# Autodesk Inventor assembly: Assembly1
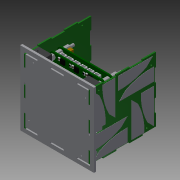
[picture p0: Inventor's stored thumbnail of the model, 180x180]
Saved by Autodesk Inventor 2015 SP1 (Build 190203100, 203)
## iProperties
Created: 2015-08-25
Part Number: Assembly1
Document SubType Name: Assembly
Designer: Kartikye
Author: Kartikye
## Documents named in this file (11)
- C:\Users\Kartikye\Documents\GitHub\SASSat\Structure\V5\Assembly1.iam
- C:\Users\Kartikye\Documents\GitHub\SASSat\Structure\V5\Bottom Panel.ipt
- C:\Users\Kartikye\Documents\GitHub\SASSat\Structure\V5\Corner2.ipt
- C:\Users\Kartikye\Documents\GitHub\SASSat\Structure\V5\Side Solar Panel.iam
- C:\Users\Kartikye\Documents\GitHub\SASSat\Structure\Imported Components\D2MQ_1\D2MQ_1.iam
- C:\Users\Kartikye\Documents\GitHub\SASSat\Structure\V5\Side Solar Panel with Switch.iam
- C:\Users\Kartikye\Documents\GitHub\SASSat\Structure\V5\Corner Switch Holder.ipt
- C:\Users\Kartikye\Documents\GitHub\SASSat\Structure\EPS\PQ60 EPS FV4.brd.iam
- C:\Users\Kartikye\Documents\GitHub\SASSat\Structure\Standoff.ipt
- C:\Users\Kartikye\Documents\GitHub\SASSat\Structure\Radio\PQ60 Radio FV1.brd.iam
- C:\Users\Kartikye\Documents\GitHub\SASSat\Structure\m1.6.ipt
## Components (31 placed, 10 different names)
1. Bottom Panel:1 — Mate:25, Mate:26, Mate:27, Mate:28, Mate:29, Mate:30, Mate:31, Mate:38, Mate:40
2. Corner Switch Holder:2 — Mate:26, Mate:36, Mate:37, Insert:1, Insert:16
3. Corner2:2 — Mate:28, Mate:34, Mate:35, Insert:2
4. Corner Switch Holder:1 — Mate:29, Mate:32, Mate:33, Mate:42, Insert:18, Insert:19
5. Corner2:4 — Mate:23, Mate:24, Mate:27, Insert:5
6. Side Solar Panel:1 [sub-assembly] — Mate:13, Mate:14, Flush:1, Mate:15, Mate:16, Flush:2, Mate:32, Mate:34
7. Side Solar Panel with Switch:2 [sub-assembly] — Mate:15, Mate:16, Flush:2, Mate:17, Mate:18, Mate:19, Flush:3, Mate:24, Mate:33, Flush:5, Mate:41, Insert:22
8. Side Solar Panel:3 [sub-assembly] — Mate:17, Mate:18, Mate:19, Flush:3, Mate:23, Mate:25, Mate:30, Mate:36
9. Side Solar Panel with Switch:1 [sub-assembly] — Mate:13, Mate:14, Flush:1, Mate:31, Mate:35, Mate:37, Mate:39, Flush:4, Insert:20
10. D2MQ_1:1 [sub-assembly] — Mate:38, Mate:39, Flush:4, Insert:21
11. D2MQ_1:2 [sub-assembly] — Mate:40, Flush:5, Mate:41
12. PQ60 EPS FV4.brd:1 [sub-assembly] — Insert:3, Insert:4, Insert:6, Insert:7, Insert:8, Insert:9
13. Standoff:1 — Insert:8
14. Standoff:2 — Insert:9, Insert:11
15. Standoff:3 — Insert:1
16. Standoff:4 — Insert:5
17. Standoff:5 — Mate:42, Insert:4
18. Standoff:6 — Insert:6
19. Standoff:7 — Insert:7, Insert:10
20. Standoff:8 — Insert:2, Insert:3
21. PQ60 Radio FV1.brd:1 [sub-assembly] — Insert:10, Insert:11, Insert:12, Insert:13, Insert:14, Insert:15
22. Standoff:9 — Insert:12
23. Standoff:10 — Insert:15
24. Standoff:11 — Insert:13
25. Standoff:12 — Insert:14
26. m1.6:1 — Insert:19
27. m1.6:2 — Insert:18
28. m1.6:3 — Insert:21
29. m1.6:4 — Insert:16
30. m1.6:5 — Insert:22
31. m1.6:6 — Insert:20
## Relationships (53: Mate 27, Insert 21, Flush 5)
- Mate:13: Side Solar Panel:1 ↔ Side Solar Panel with Switch:1
- Mate:14: Side Solar Panel:1 ↔ Side Solar Panel with Switch:1
- Flush:1: Side Solar Panel:1 ↔ Side Solar Panel with Switch:1
- Mate:15: Side Solar Panel:1 ↔ Side Solar Panel with Switch:2
- Mate:16: Side Solar Panel:1 ↔ Side Solar Panel with Switch:2
- Flush:2: Side Solar Panel:1 ↔ Side Solar Panel with Switch:2
- Mate:17: Side Solar Panel with Switch:2 ↔ Side Solar Panel:3
- Mate:18: Side Solar Panel with Switch:2 ↔ Side Solar Panel:3
- Mate:19: Side Solar Panel with Switch:2 ↔ Side Solar Panel:3
- Flush:3: Side Solar Panel with Switch:2 ↔ Side Solar Panel:3
- Mate:23: Corner2:4 ↔ Side Solar Panel:3
- Mate:24: Corner2:4 ↔ Side Solar Panel with Switch:2
- Mate:25: Bottom Panel:1 ↔ Side Solar Panel:3
- Mate:26: Bottom Panel:1 ↔ Corner Switch Holder:2
- Mate:27: Bottom Panel:1 ↔ Corner2:4
- Mate:28: Bottom Panel:1 ↔ Corner2:2
- Mate:29: Bottom Panel:1 ↔ Corner Switch Holder:1
- Mate:30: Bottom Panel:1 ↔ Side Solar Panel:3
- Mate:31: Bottom Panel:1 ↔ Side Solar Panel with Switch:1
- Mate:32: Corner Switch Holder:1 ↔ Side Solar Panel:1
- Mate:33: Corner Switch Holder:1 ↔ Side Solar Panel with Switch:2
- Mate:34: Corner2:2 ↔ Side Solar Panel:1
- Mate:35: Corner2:2 ↔ Side Solar Panel with Switch:1
- Mate:36: Corner Switch Holder:2 ↔ Side Solar Panel:3
- Mate:37: Corner Switch Holder:2 ↔ Side Solar Panel with Switch:1
- Mate:38: Bottom Panel:1 ↔ D2MQ_1:1
- Mate:39: Side Solar Panel with Switch:1 ↔ D2MQ_1:1
- Flush:4: Side Solar Panel with Switch:1 ↔ D2MQ_1:1
- Mate:40: Bottom Panel:1 ↔ D2MQ_1:2
- Flush:5: Side Solar Panel with Switch:2 ↔ D2MQ_1:2
- Mate:41: Side Solar Panel with Switch:2 ↔ D2MQ_1:2
- Insert:1: Corner Switch Holder:2 ↔ Standoff:3
- Insert:2: Corner2:2 ↔ Standoff:8
- Mate:42: Corner Switch Holder:1 ↔ Standoff:5
- Insert:3: PQ60 EPS FV4.brd:1 ↔ Standoff:8
- Insert:4: PQ60 EPS FV4.brd:1 ↔ Standoff:5
- Insert:5: Corner2:4 ↔ Standoff:4
- Insert:6: PQ60 EPS FV4.brd:1 ↔ Standoff:6
- Insert:7: PQ60 EPS FV4.brd:1 ↔ Standoff:7
- Insert:8: PQ60 EPS FV4.brd:1 ↔ Standoff:1
- Insert:9: PQ60 EPS FV4.brd:1 ↔ Standoff:2
- Insert:10: Standoff:7 ↔ PQ60 Radio FV1.brd:1
- Insert:11: Standoff:2 ↔ PQ60 Radio FV1.brd:1
- Insert:12: PQ60 Radio FV1.brd:1 ↔ Standoff:9
- Insert:13: PQ60 Radio FV1.brd:1 ↔ Standoff:11
- Insert:14: PQ60 Radio FV1.brd:1 ↔ Standoff:12
- Insert:15: PQ60 Radio FV1.brd:1 ↔ Standoff:10
- Insert:16: Corner Switch Holder:2 ↔ m1.6:4
- Insert:18: Corner Switch Holder:1 ↔ m1.6:2
- Insert:19: Corner Switch Holder:1 ↔ m1.6:1
- Insert:20: Side Solar Panel with Switch:1 ↔ m1.6:6
- Insert:21: D2MQ_1:1 ↔ m1.6:3
- Insert:22: Side Solar Panel with Switch:2 ↔ m1.6:5
